# Autodesk Inventor assembly: assemble_ver3_prod
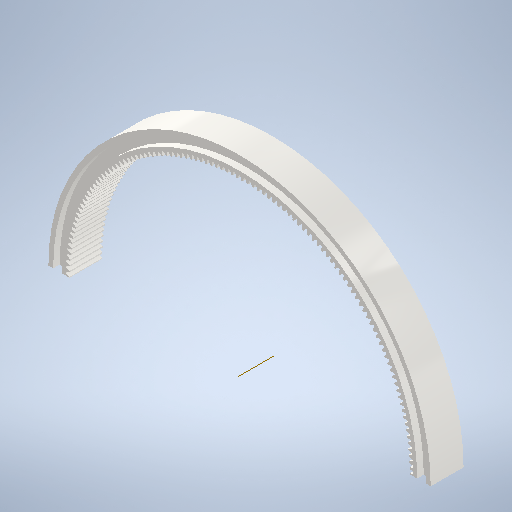
[picture p0: Inventor's stored thumbnail of the model, 512x512]
Saved by Autodesk Inventor 2025 (Build 290162000, 162)
## iProperties
Created: 2025-10-01
Part Number: assemble_ver3_prod
Document SubType Name: Assembly
Designer: Admin
Author: Admin
## Documents named in this file (3)
- C:\Users\sum89\OneDrive\Рабочий стол\Ring\Model\assemble_ver3_prod.iam
- C:\Users\sum89\OneDrive\Рабочий стол\Ring\Model\assemble_ver3\Мастер проектирования\Цилиндрическое зубчатое зацепление2.iam
- C:\Users\sum89\OneDrive\Рабочий стол\Ring\Model\Inner_main_ver3.ipt
## Components (2 placed, 2 different names)
1. Цилиндрическое зубчатое зацепление:1 [sub-assembly] — Совмещение:1, Заподлицо:1
2. Inner_main_ver3:1
## Relationships (2: Mate 1, Flush 1)
- Совмещение:1 [Mate]: Цилиндрическое зубчатое зацепление:1
- Заподлицо:1 [Flush] (-10 mm): Цилиндрическое зубчатое зацепление:1
